# Autodesk Inventor assembly: Assembly1
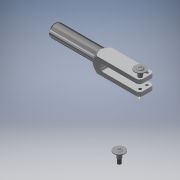
[picture p0: Inventor's stored thumbnail of the model, 180x180]
Saved by Autodesk Inventor 2017 (Build 210142000, 142)
## iProperties
Created: 2017-04-18
Part Number: Assembly1
Document SubType Name: Assembly
Designer: 193515
Author: 193515
## Documents named in this file (9)
- C:\Users\193515.FCBOE.000\Desktop\8.1\Assembly1.iam
- C:\Users\193515.FCBOE.000\Desktop\8.1\handle bar.ipt
- C:\Users\193515.FCBOE.000\Desktop\8.1\inch screw piece.ipt
- C:\Users\193515.FCBOE.000\Desktop\8.1\middle handle piece (hard) (1).ipt
- C:\Users\193515.FCBOE.000\Desktop\8.1\Part2.ipt
- C:\Users\193515.FCBOE.000\Desktop\8.1\star head screw.ipt
- C:\Users\193515.FCBOE.000\Desktop\8.1\long washer.ipt
- C:\Users\193515.FCBOE.000\Desktop\8.1\normal washer.ipt
- C:\Users\193515.FCBOE.000\Desktop\8.1\thin washer.ipt
## Components (12 placed, 8 different names)
1. handle bar:1 — Slider:1
2. inch screw piece:1 — Rigid:1
3. middle handle piece (hard) (1):1 — Rotational:1, Slider:1, Rigid:1, Rotational:5
4. Part2:1 — Rotational:1
5. star head screw:1 — Rotational:2
6. long washer:1 — Rotational:4, Rotational:5
7. normal washer:1 — Rotational:3, Rotational:4
8. thin washer:1 — Rotational:2, Rotational:3
9. long washer:2 — Rotational:7
10. normal washer:2 — Rigid:2, Rotational:7
11. star head screw:2 — Rotational:6, Rigid:2
12. thin washer:2 — Rotational:6
## Relationships (10: RevoluteJoint 7, WeldJoint 2, TranslationJoint 1)
- Rotational:1 [RevoluteJoint]: middle handle piece (hard) (1):1 ↔ Part2:1
- Slider:1 [TranslationJoint] (-1.5875 mm): handle bar:1 ↔ middle handle piece (hard) (1):1
- Rigid:1 [WeldJoint]: inch screw piece:1 ↔ middle handle piece (hard) (1):1
- Rotational:2 [RevoluteJoint]: star head screw:1 ↔ thin washer:1
- Rotational:3 [RevoluteJoint]: normal washer:1 ↔ thin washer:1
- Rotational:4 [RevoluteJoint]: long washer:1 ↔ normal washer:1
- Rotational:5 [RevoluteJoint]: middle handle piece (hard) (1):1 ↔ long washer:1
- Rotational:6 [RevoluteJoint]: star head screw:2 ↔ thin washer:2
- Rigid:2 [WeldJoint]: normal washer:2 ↔ star head screw:2
- Rotational:7 [RevoluteJoint]: long washer:2 ↔ normal washer:2
